# Autodesk Inventor assembly: CoreXY_A
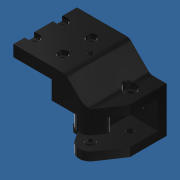
[picture p0: Inventor's stored thumbnail of the model, 180x180]
Saved by Autodesk Inventor 2020 (Build 240168000, 168)
## iProperties
Created: 2021-07-10
Part Number: CoreXY_A
Document SubType Name: Assembly
Designer: ken113
Author: ken113
## Documents named in this file (3)
- D:\Document\Github\Cheap_Belt_Printer\Model\Parts\Print_Parts\Print_Asem\CoreXY_A.iam
- D:\Document\Github\Cheap_Belt_Printer\Model\Parts\Print_Parts\Print_Parts_A_rev2.ipt
- D:\Document\Github\Cheap_Belt_Printer\Model\Parts\Print_Parts\Print_Parts_B_rev2.ipt
## Components (2 placed, 2 different names)
1. Print_Parts_A_rev2:1 — フラッシュ:1, メイト:2, フラッシュ:2
2. Print_Parts_B_rev2:1 — フラッシュ:1, メイト:2, フラッシュ:2
## Relationships (3: Flush 2, Mate 1)
- フラッシュ:1 [Flush]: Print_Parts_A_rev2:1 ↔ Print_Parts_B_rev2:1
- メイト:2 [Mate]: Print_Parts_A_rev2:1 ↔ Print_Parts_B_rev2:1
- フラッシュ:2 [Flush]: Print_Parts_A_rev2:1 ↔ Print_Parts_B_rev2:1
